# Autodesk Inventor assembly: 1756-211
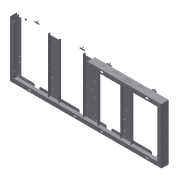
[picture p0: Inventor's stored thumbnail of the model, 180x180]
Saved by Autodesk Inventor 2017 (Build 210142000, 142)
## iProperties
Created: 2014-02-17
Part Number: 1756-211
Document SubType Name: Assembly
Designer: Евтушенко
Author: Евтушенко
## Documents named in this file (6)
- D:\ИНИТ\STEP файлы\Колонки\OCEAN-36-WAVE\1756-211.iam
- D:\ИНИТ\STEP файлы\Колонки\OCEAN-36-WAVE\1756-211-01.ipt
- D:\ИНИТ\STEP файлы\Колонки\OCEAN-36-WAVE\1756-211-02.ipt
- D:\ИНИТ\STEP файлы\Колонки\OCEAN-36-WAVE\1756-211-03.iam
- D:\ИНИТ\STEP файлы\Колонки\OCEAN-36-WAVE\Matice_privarovaci_DIN-929_M8.ipt
- D:\ИНИТ\STEP файлы\Колонки\OCEAN-36-WAVE\Matice_privarovaci_DIN-929_M6.ipt
## Components (15 placed, 5 different names)
1. 1756-211-01:1 — Заподлицо:1, Совмещение:1
2. 1756-211-02:1 — Заподлицо:1, Совмещение:1
3. 1756-211-03:1 [sub-assembly]
4. Matice_privarovaci_DIN-929_M8:1
5. Matice_privarovaci_DIN-929_M8:3
6. Matice_privarovaci_DIN-929_M8:4
7. Matice_privarovaci_DIN-929_M6:1
8. Matice_privarovaci_DIN-929_M6:2
9. Matice_privarovaci_DIN-929_M8:12
10. Matice_privarovaci_DIN-929_M8:13
11. Matice_privarovaci_DIN-929_M8:14
12. Matice_privarovaci_DIN-929_M6:3
13. Matice_privarovaci_DIN-929_M6:4
14. Matice_privarovaci_DIN-929_M8:15
15. Matice_privarovaci_DIN-929_M8:16
## Relationships (2: Flush 1, Mate 1)
- Заподлицо:1 [Flush]: 1756-211-01:1 ↔ 1756-211-02:1
- Совмещение:1 [Mate] (-520 mm): 1756-211-01:1 ↔ 1756-211-02:1
